# Autodesk Inventor assembly: Z-Axis Transmission Assembly Back
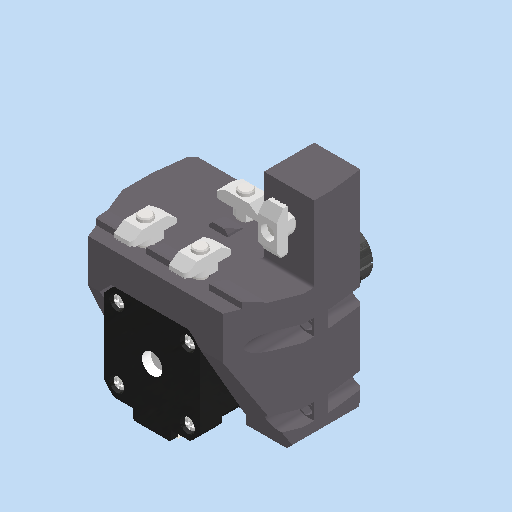
[picture p0: Inventor's stored thumbnail of the model, 512x512]
Saved by Autodesk Inventor 2023.2 (Build 272271000, 271)
## iProperties
Created: 2023-11-27
Part Number: Z-Axis Transmission Assembly Back
Document SubType Name: Assembly
Designer: Nils Bade
Author: Nils Bade
## Documents named in this file (10)
- C:\Users\nilsb\Documents\Inventor\Projektarbeit-Bade\RatRig_Bade\Z-Axis Transmission Assembly Back.iam
- C:\Users\nilsb\Documents\Inventor\Projektarbeit-Bade\RatRig_modified\Leadscrew Motorcage Back for 4040.ipt
- C:\Users\nilsb\Documents\Inventor\Projektarbeit-Bade\RatRig_Standards\Nema 17 Stepper Motor - 48mm - 1.8degree_step, 76oz-in v1.ipt
- C:\Users\nilsb\Documents\Inventor\Projektarbeit-Bade\RatRig_Standards\pillow_block v2.ipt
- C:\Users\nilsb\Documents\Inventor\Projektarbeit-Bade\RatRig_Standards\Thrust Bearing F8-16M v1.ipt
- C:\Users\nilsb\Documents\Inventor\Projektarbeit-Bade\RatRig_Standards\Coupler - Rigid Type - Black 25x20mm - 5mm to 8mm v2.iam
- C:\Users\nilsb\Documents\Inventor\Projektarbeit-Bade\Schrauben\Cap Head Screw M3x18 v2.ipt
- C:\Users\nilsb\Documents\Inventor\Projektarbeit-Bade\RatRig_modified\T-NUT - DropIn 4040 SERIES - M6.ipt
- C:\Users\nilsb\Documents\Inventor\Projektarbeit-Bade\Schrauben\Cap Head Screw M6x20 v2.ipt
- C:\Users\nilsb\Documents\Inventor\Projektarbeit-Bade\Schrauben\Cap Head Screw M6x16.ipt
## Components (17 placed, 9 different names)
1. Lead Screw Motor Cage Back for 4040:1 — Passend:1, Winkel:1, Passend:2, Passend:4, Passend:5, Passend:6, Passend:18, Passend:19, Passend:20, Winkel:3, Winkel:4, Winkel:5, Winkel:6, Passend:21, Passend:25, Passend:29, Passend:30, Passend:31, Passend:32, Passend:33, Passend:34, Passend:35, Passend:36, Passend:37, Passend:38, Passend:39
2. Nema 17 Stepper Motor - 48mm - 1.8degree_step, 76oz-in v1:1 — Passend:1, Winkel:1, Passend:2, Passend:3, Passend:8
3. pillow_block v2:1 — Passend:4, Passend:5, Passend:6, Passend:7, Winkel:2, Passend:10, Passend:11, Passend:12, Passend:13, Passend:14, Passend:15, Passend:16, Passend:17
4. Thrust Bearing F8-16M v1:1 — Passend:3, Passend:7, Passend:9
5. Coupler - Rigid Type - Black 25x20mm - 5mm to 8mm v2:1 [sub-assembly] — Passend:8, Passend:9, Winkel:2
6. Cap Head Screw M3x18 v2:1 — Passend:10, Passend:14
7. Cap Head Screw M3x18 v2:2 — Passend:12, Passend:16
8. Cap Head Screw M3x18 v2:3 — Passend:11, Passend:15
9. Cap Head Screw M3x18 v2:4 — Passend:13, Passend:17
10. T-NUT - DROP IN TYPE FOR 40 SERIES - M6:1 — Passend:18, Winkel:3, Passend:29
11. T-NUT - DROP IN TYPE FOR 40 SERIES - M6:2 — Passend:19, Winkel:4, Passend:30
12. T-NUT - DROP IN TYPE FOR 40 SERIES - M6:3 — Passend:20, Winkel:5, Passend:31
13. T-NUT - DROP IN TYPE FOR 40 SERIES - M6:4 — Winkel:6, Passend:21, Passend:32
14. Cap Head Screw M6x20 v2:1 — Passend:25, Passend:33
15. Cap Head Screw M6x16:1 — Passend:34, Passend:39
16. Cap Head Screw M6x16:2 — Passend:35, Passend:38
17. Cap Head Screw M6x16:3 — Passend:36, Passend:37
## Relationships (39: Mate 33, Angle 6)
- Passend:1 [Mate]: Lead Screw Motor Cage Back for 4040:1 ↔ Nema 17 Stepper Motor - 48mm - 1.8degree_step, 76oz-in v1:1
- Winkel:1 [Angle] (180 deg): Lead Screw Motor Cage Back for 4040:1 ↔ Nema 17 Stepper Motor - 48mm - 1.8degree_step, 76oz-in v1:1
- Passend:2 [Mate]: Lead Screw Motor Cage Back for 4040:1 ↔ Nema 17 Stepper Motor - 48mm - 1.8degree_step, 76oz-in v1:1
- Passend:3 [Mate]: Nema 17 Stepper Motor - 48mm - 1.8degree_step, 76oz-in v1:1 ↔ Thrust Bearing F8-16M v1:1
- Passend:4 [Mate]: Lead Screw Motor Cage Back for 4040:1 ↔ pillow_block v2:1
- Passend:5 [Mate]: Lead Screw Motor Cage Back for 4040:1 ↔ pillow_block v2:1
- Passend:6 [Mate]: Lead Screw Motor Cage Back for 4040:1 ↔ pillow_block v2:1
- Passend:7 [Mate]: pillow_block v2:1 ↔ Thrust Bearing F8-16M v1:1
- Passend:8 [Mate]: Nema 17 Stepper Motor - 48mm - 1.8degree_step, 76oz-in v1:1 ↔ Coupler - Rigid Type - Black 25x20mm - 5mm to 8mm v2:1
- Passend:9 [Mate]: Thrust Bearing F8-16M v1:1 ↔ Coupler - Rigid Type - Black 25x20mm - 5mm to 8mm v2:1
- Winkel:2 [Angle] (90 deg): pillow_block v2:1 ↔ Coupler - Rigid Type - Black 25x20mm - 5mm to 8mm v2:1
- Passend:10 [Mate]: pillow_block v2:1 ↔ Cap Head Screw M3x18 v2:1
- Passend:11 [Mate]: pillow_block v2:1 ↔ Cap Head Screw M3x18 v2:3
- Passend:12 [Mate]: pillow_block v2:1 ↔ Cap Head Screw M3x18 v2:2
- Passend:13 [Mate]: pillow_block v2:1 ↔ Cap Head Screw M3x18 v2:4
- Passend:14 [Mate]: pillow_block v2:1 ↔ Cap Head Screw M3x18 v2:1
- Passend:15 [Mate]: pillow_block v2:1 ↔ Cap Head Screw M3x18 v2:3
- Passend:16 [Mate]: pillow_block v2:1 ↔ Cap Head Screw M3x18 v2:2
- Passend:17 [Mate]: pillow_block v2:1 ↔ Cap Head Screw M3x18 v2:4
- Passend:18 [Mate]: Lead Screw Motor Cage Back for 4040:1 ↔ T-NUT - DROP IN TYPE FOR 40 SERIES - M6:1
- Passend:19 [Mate]: Lead Screw Motor Cage Back for 4040:1 ↔ T-NUT - DROP IN TYPE FOR 40 SERIES - M6:2
- Passend:20 [Mate]: Lead Screw Motor Cage Back for 4040:1 ↔ T-NUT - DROP IN TYPE FOR 40 SERIES - M6:3
- Winkel:3 [Angle] (90 deg): Lead Screw Motor Cage Back for 4040:1 ↔ T-NUT - DROP IN TYPE FOR 40 SERIES - M6:1
- Winkel:4 [Angle] (0 deg): Lead Screw Motor Cage Back for 4040:1 ↔ T-NUT - DROP IN TYPE FOR 40 SERIES - M6:2
- Winkel:5 [Angle] (0 deg): Lead Screw Motor Cage Back for 4040:1 ↔ T-NUT - DROP IN TYPE FOR 40 SERIES - M6:3
- Winkel:6 [Angle] (0 deg): Lead Screw Motor Cage Back for 4040:1 ↔ T-NUT - DROP IN TYPE FOR 40 SERIES - M6:4
- Passend:21 [Mate]: Lead Screw Motor Cage Back for 4040:1 ↔ T-NUT - DROP IN TYPE FOR 40 SERIES - M6:4
- Passend:25 [Mate]: Lead Screw Motor Cage Back for 4040:1 ↔ Cap Head Screw M6x20 v2:1
- Passend:29 [Mate] (4.5 mm): Lead Screw Motor Cage Back for 4040:1 ↔ T-NUT - DROP IN TYPE FOR 40 SERIES - M6:1
- Passend:30 [Mate] (4.5 mm): Lead Screw Motor Cage Back for 4040:1 ↔ T-NUT - DROP IN TYPE FOR 40 SERIES - M6:2
- Passend:31 [Mate] (4.5 mm): Lead Screw Motor Cage Back for 4040:1 ↔ T-NUT - DROP IN TYPE FOR 40 SERIES - M6:3
- Passend:32 [Mate] (4.5 mm): Lead Screw Motor Cage Back for 4040:1 ↔ T-NUT - DROP IN TYPE FOR 40 SERIES - M6:4
- Passend:33 [Mate]: Lead Screw Motor Cage Back for 4040:1 ↔ Cap Head Screw M6x20 v2:1
- Passend:34 [Mate]: Lead Screw Motor Cage Back for 4040:1 ↔ Cap Head Screw M6x16:1
- Passend:35 [Mate]: Lead Screw Motor Cage Back for 4040:1 ↔ Cap Head Screw M6x16:2
- Passend:36 [Mate]: Lead Screw Motor Cage Back for 4040:1 ↔ Cap Head Screw M6x16:3
- Passend:37 [Mate]: Lead Screw Motor Cage Back for 4040:1 ↔ Cap Head Screw M6x16:3
- Passend:38 [Mate]: Lead Screw Motor Cage Back for 4040:1 ↔ Cap Head Screw M6x16:2
- Passend:39 [Mate]: Lead Screw Motor Cage Back for 4040:1 ↔ Cap Head Screw M6x16:1
